# Autodesk Inventor assembly: Arm
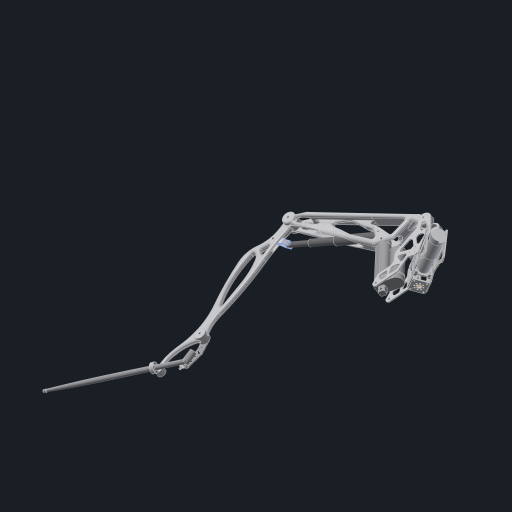
[picture p0: Inventor's stored thumbnail of the model, 512x512]
Saved by Autodesk Inventor 2023 (Build 270158000, 158)
## iProperties
Created: 2020-03-24
Part Number: Arm
Document SubType Name: Assembly
Designer: valer
Mass: 4853.13 g
Surface Area: 3141.52 cm^2
Volume: 1403.99 cm^3
Density: 3.45667 g/cm^3
Author: valer
## Documents named in this file (12)
- C:\Users\valer\Desktop\str1ker\cad\Arm.iam
- C:\Users\valer\Desktop\str1ker\cad\ArmBase.iam
- C:\Users\valer\Desktop\str1ker\cad\Shoulder.iam
- C:\Users\valer\Desktop\str1ker\cad\UpperArm.iam
- C:\Users\valer\Desktop\str1ker\cad\Forearm.iam
- C:\Users\valer\Desktop\str1ker\cad\Drumstick.iam
- C:\Users\valer\Desktop\str1ker\cad\ArmSolenoid.iam
- C:\Users\valer\Desktop\str1ker\cad\external\UpperArmActuator\UpperArmActuatorBase.iam
- C:\Users\valer\Desktop\str1ker\cad\external\UpperArmActuator\UpperArmActuatorShaft.iam
- C:\Users\valer\Desktop\str1ker\cad\external\ForearmActuator\ForearmActuatorBody.iam
- C:\Users\valer\Desktop\str1ker\cad\external\ForearmActuator\ForearmActuatorShaft.iam
- C:\Users\valer\Desktop\str1ker\cad\ForearmActuatorConnector.iam
## Components (11 placed, 11 different names)
1. Base:1 [sub-assembly] — Flush:1, Flush:2, Mate:1, Mate:2, Mate:3
2. Shoulder:1 [sub-assembly] — Mate:1, Mate:2, Mate:4, Mate:5, Mate:12, Mate:15
3. UpperArm:1 [sub-assembly] — Mate:4, Mate:5, Mate:6, Mate:7, Mate:13, Mate:17
4. Forearm:1 [sub-assembly] — Mate:6, Mate:7, Mate:8, Mate:9, Mate:10, Mate:11, Mate:19, Mate:21
5. Drumstick:1 [sub-assembly] — Mate:8, Mate:9
6. ArmSolenoid:1 [sub-assembly] — Mate:10, Mate:11
7. UpperArmActuatorBase:1 [sub-assembly] — Mate:12, Mate:14, Mate:15
8. UpperArmActuatorShaft:1 [sub-assembly] — Mate:13, Mate:14
9. ForearmActuatorBody:1 [sub-assembly] — Mate:16, Mate:17
10. ForearmActuatorShaft:1 [sub-assembly] — Mate:16, Mate:18, Mate:20
11. ForearmActuatorConnector:1 [sub-assembly] — Mate:18, Mate:19, Mate:20, Mate:21
## Relationships (23: Mate 21, Flush 2)
- Flush:1: Base:1
- Flush:2: Base:1
- Mate:1: Base:1 ↔ Shoulder:1
- Mate:2: Base:1 ↔ Shoulder:1
- Mate:3: Base:1
- Mate:4: Shoulder:1 ↔ UpperArm:1
- Mate:5: Shoulder:1 ↔ UpperArm:1
- Mate:6: UpperArm:1 ↔ Forearm:1
- Mate:7: UpperArm:1 ↔ Forearm:1
- Mate:8: Forearm:1 ↔ Drumstick:1
- Mate:9: Forearm:1 ↔ Drumstick:1
- Mate:10: Forearm:1 ↔ ArmSolenoid:1
- Mate:11: Forearm:1 ↔ ArmSolenoid:1
- Mate:12: Shoulder:1 ↔ UpperArmActuatorBase:1
- Mate:13: UpperArm:1 ↔ UpperArmActuatorShaft:1
- Mate:14: UpperArmActuatorBase:1 ↔ UpperArmActuatorShaft:1
- Mate:15 (11 mm): Shoulder:1 ↔ UpperArmActuatorBase:1
- Mate:16: ForearmActuatorBody:1 ↔ ForearmActuatorShaft:1
- Mate:17: UpperArm:1 ↔ ForearmActuatorBody:1
- Mate:18: ForearmActuatorShaft:1 ↔ ForearmActuatorConnector:1
- Mate:19: Forearm:1 ↔ ForearmActuatorConnector:1
- Mate:20: ForearmActuatorShaft:1 ↔ ForearmActuatorConnector:1
- Mate:21: Forearm:1 ↔ ForearmActuatorConnector:1
